# Autodesk Inventor assembly: Сборка4
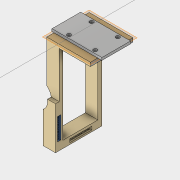
[picture p0: Inventor's stored thumbnail of the model, 180x180]
Saved by Autodesk Inventor 2021.2 (Build 252289000, 289)
## iProperties
Created: 2025-10-29
Part Number: Сборка4
Document SubType Name: Assembly
Designer: Захаров
Author: Захаров
## Documents named in this file (3)
- C:\Users\User\Documents\ARHeadGen1\Сборка4.iam
- C:\Users\User\Documents\ARHeadGen1\ЛЦМК000002.00.00.00.00.06-02.ipt
- C:\Users\User\Documents\ARHeadGen1\ЛЦМК000002.00.00.00.00.11.ipt
## Components (2 placed, 2 different names)
1. ЛЦМК000002.00.00.00.00.06-02:1 — Совмещение:1, Совмещение:2, Совмещение:3
2. ЛЦМК000002.00.00.00.00.11:1 — Совмещение:1, Совмещение:2, Совмещение:3
## Relationships (3: Mate 3)
- Совмещение:1 [Mate]: ЛЦМК000002.00.00.00.00.06-02:1 ↔ ЛЦМК000002.00.00.00.00.11:1
- Совмещение:2 [Mate]: ЛЦМК000002.00.00.00.00.06-02:1 ↔ ЛЦМК000002.00.00.00.00.11:1
- Совмещение:3 [Mate]: ЛЦМК000002.00.00.00.00.06-02:1 ↔ ЛЦМК000002.00.00.00.00.11:1
